# Autodesk Inventor assembly: 16631023
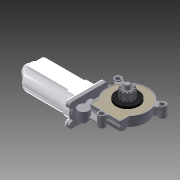
[picture p0: Inventor's stored thumbnail of the model, 180x180]
Saved by Autodesk Inventor 2014 (Build 180170000, 170)
## iProperties
Category: Motors
Company: Autodesk, Inc.
Created: 2013-12-31
Part Number: 16631023
Document SubType Name: Assembly
Project: FIRST
Description: Motor - Keyang LH 12 tooth pinion
Vendor: Keyang
Mass: 850 g
Surface Area: 430.457 cm^2
Volume: 226.7 cm^3
Catalog Web Link: http://www.usfirst.org/uploadedFiles/Community/FRC/FRC_Documents_and_Updates/2008_Assets/Manual/Keyang%20Motor%20Specs%20-%2016627960%20and%2061.pdf
Designer: Autodesk, Inc.
Title: Motor - Keyang LH 12 tooth pinion
Author: Autodesk, Inc.
## Documents named in this file (3)
- D:\Data Folder\FIRST 2014\KOP Parts\Motors\MOT_Keyang_16631023.iam
- D:\Data Folder\FIRST 2014\KOP Parts\Motors\Parts\16631023_body_LH.ipt
- D:\Data Folder\FIRST 2014\KOP Parts\Motors\Parts\16631023_12 tooth pinion gear.ipt
## Components (2 placed, 2 different names)
1. 16631023_body_LH:1 — Mate:1
2. 16631023_12 tooth pinion gear:1 — Mate:1
## Relationships (2: Mate 2)
- Mate:1: 16631023_body_LH:1 ↔ 16631023_12 tooth pinion gear:1
- [Mate]: 16631023_body_LH:1 ↔ 16631023_12 tooth pinion gear:1
